# Autodesk Inventor assembly: A2017_T2_07
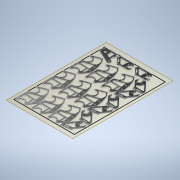
[picture p0: Inventor's stored thumbnail of the model, 180x180]
Saved by Autodesk Inventor 2022.3 (Build 263350000, 350)
## iProperties
Created: 2022-09-28
Part Number: A2017_T2_07
Document SubType Name: Assembly
Designer: Masato
Author: Masato
## Documents named in this file (5)
- C:\Users\Masato\Documents\Inventor\Inventor for CIT Brains\SUSTAINA-OP - cam\Cam\A2017_T2\A2017_T2_07.iam
- C:\Users\Masato\Documents\Inventor\Inventor for CIT Brains\SUSTAINA-OP - cam\Cam\DisposableBoard.ipt
- C:\Users\Masato\Documents\Inventor\Inventor for CIT Brains\SUSTAINA-OP - cam\LowerBody\Knee\Knee_side_frame.ipt
- C:\Users\Masato\Documents\Inventor\Inventor for CIT Brains\SUSTAINA-OP - cam\UpperBody\Arm\Shoulder_side_frame.ipt
- C:\Users\Masato\Documents\Inventor\Inventor for CIT Brains\SUSTAINA-OP - cam\LowerBody\Leg_joint\Leg_joint_pitch_frame.ipt
## Components (19 placed, 4 different names)
1. DisposableBoard:1 — フラッシュ:1, フラッシュ:2, フラッシュ:3, フラッシュ:4, 角度:1, 正接:1, フラッシュ:6, 正接:4, フラッシュ:9, 正接:8, フラッシュ:7, フラッシュ:8
2. Leg_joint_pitch_frame:1 — メイト:8, フラッシュ:7, フラッシュ:8, メイト:9
3. Knee_side_frame:1 — メイト:2, 角度:1, 正接:1, フラッシュ:6
4. Knee_side_frame:2
5. Knee_side_frame:3
6. Knee_side_frame:4
7. Knee_side_frame:5
8. Knee_side_frame:6
9. Knee_side_frame:7 — メイト:3, 正接:7, 正接:3
10. Knee_side_frame:8
11. Knee_side_frame:9
12. Shoulder_side_frame:5 — メイト:7, フラッシュ:9, メイト:9
13. Shoulder_side_frame:6
14. Shoulder_side_frame:1 — メイト:3, メイト:5, 正接:7, 正接:2, 正接:8
15. Shoulder_side_frame:3 — メイト:4, 正接:2, 正接:3, 正接:4
16. Shoulder_side_frame:9
17. Shoulder_side_frame:10
18. Shoulder_side_frame:11
19. Shoulder_side_frame:12
## Component patterns: (9 elements, first: Knee_side_frame:1), (2 elements, first: Shoulder_side_frame:5), (3 elements, first: Shoulder_side_frame:1 + Shoulder_side_frame:3)
## Relationships (22: Flush 8, Mate 7, Tangent 6, Angle 1)
- フラッシュ:1 [Flush]: DisposableBoard:1
- フラッシュ:2 [Flush]: DisposableBoard:1
- フラッシュ:3 [Flush]: DisposableBoard:1
- フラッシュ:4 [Flush]: DisposableBoard:1
- メイト:2 [Mate]: Knee_side_frame:1
- 角度:1 [Angle] (0 deg): DisposableBoard:1 ↔ Knee_side_frame:1
- 正接:1 [Tangent] (2 mm): DisposableBoard:1 ↔ Knee_side_frame:1
- メイト:3 [Mate]: Knee_side_frame:7 ↔ Shoulder_side_frame:1
- フラッシュ:6 [Flush] (-2 mm): DisposableBoard:1 ↔ Knee_side_frame:1
- メイト:4 [Mate]: Shoulder_side_frame:3
- メイト:5 [Mate]: Shoulder_side_frame:1
- 正接:7 [Tangent] (2.1 mm): Knee_side_frame:7 ↔ Shoulder_side_frame:1
- 正接:2 [Tangent] (2.1 mm): Shoulder_side_frame:1 ↔ Shoulder_side_frame:3
- 正接:3 [Tangent] (2.1 mm): Knee_side_frame:7 ↔ Shoulder_side_frame:3
- 正接:4 [Tangent] (2 mm): DisposableBoard:1 ↔ Shoulder_side_frame:3
- メイト:7 [Mate]: Shoulder_side_frame:5
- フラッシュ:9 [Flush] (2.1 mm): DisposableBoard:1 ↔ Shoulder_side_frame:5
- 正接:8 [Tangent] (2 mm): DisposableBoard:1 ↔ Shoulder_side_frame:1
- メイト:8 [Mate]: Leg_joint_pitch_frame:1
- フラッシュ:7 [Flush] (-2 mm): DisposableBoard:1 ↔ Leg_joint_pitch_frame:1
- フラッシュ:8 [Flush] (-2 mm): DisposableBoard:1 ↔ Leg_joint_pitch_frame:1
- メイト:9 [Mate] (2.1 mm): Leg_joint_pitch_frame:1 ↔ Shoulder_side_frame:5
